# Autodesk Inventor assembly: GFRP_T2_09
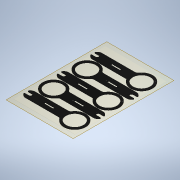
[picture p0: Inventor's stored thumbnail of the model, 180x180]
Saved by Autodesk Inventor 2020 (Build 240168000, 168)
## iProperties
Created: 2021-08-27
Part Number: GFRP_T2_09
Document SubType Name: Assembly
Designer: Masato
Author: Masato
## Documents named in this file (3)
- C:\Users\naoki\Documents\Inventor\CitBrains\git_clone\SUSTAINA_ver1_0\A_T2_175\SUSTAINA-OP\Cam\GFRP_T2_09.iam
- C:\Users\naoki\Documents\Inventor\CitBrains\git_clone\SUSTAINA_ver1_0\A_T2_175\SUSTAINA-OP\Cam\DisposableBoard.ipt
- C:\Users\naoki\Documents\Inventor\CitBrains\git_clone\SUSTAINA_ver1_0\A_T2_175\SUSTAINA-OP\UpperBody\Arm\ForeArm_outside_frame.ipt
## Components (6 placed, 2 different names)
1. DisposableBoard:1 — メイト:2, メイト:1, フラッシュ:1, フラッシュ:2, メイト:4, メイト:5, 角度:1, 正接:1, 正接:2, 正接:3, メイト:6, 正接:6
2. ForeArm_outside_frame:5 — メイト:6, 正接:5, 正接:6, 角度:3
3. ForeArm_outside_frame:1 — メイト:4, 角度:1, 角度:2, 正接:1, 正接:2, 正接:4
4. ForeArm_outside_frame:2 — メイト:5, 角度:2, 正接:3, 正接:4
5. ForeArm_outside_frame:3
6. ForeArm_outside_frame:4 — 正接:5, 角度:3
## Component patterns: (2 elements, first: ForeArm_outside_frame:1 + ForeArm_outside_frame:2)
## Relationships (16: Tangent 6, Mate 5, Angle 3, Flush 2)
- メイト:2 [Mate]: DisposableBoard:1
- メイト:1 [Mate]: DisposableBoard:1
- フラッシュ:1 [Flush]: DisposableBoard:1
- フラッシュ:2 [Flush]: DisposableBoard:1
- メイト:4 [Mate]: DisposableBoard:1 ↔ ForeArm_outside_frame:1
- メイト:5 [Mate]: DisposableBoard:1 ↔ ForeArm_outside_frame:2
- 角度:1 [Angle] (0 deg): DisposableBoard:1 ↔ ForeArm_outside_frame:1
- 角度:2 [Angle] (0 deg): ForeArm_outside_frame:1 ↔ ForeArm_outside_frame:2
- 正接:1 [Tangent] (2 mm): DisposableBoard:1 ↔ ForeArm_outside_frame:1
- 正接:2 [Tangent] (2 mm): DisposableBoard:1 ↔ ForeArm_outside_frame:1
- 正接:3 [Tangent] (2 mm): DisposableBoard:1 ↔ ForeArm_outside_frame:2
- 正接:4 [Tangent] (2.5 mm): ForeArm_outside_frame:1 ↔ ForeArm_outside_frame:2
- メイト:6 [Mate]: DisposableBoard:1 ↔ ForeArm_outside_frame:5
- 正接:5 [Tangent] (2.5 mm): ForeArm_outside_frame:5 ↔ ForeArm_outside_frame:4
- 正接:6 [Tangent] (2 mm): DisposableBoard:1 ↔ ForeArm_outside_frame:5
- 角度:3 [Angle] (0 deg): ForeArm_outside_frame:5 ↔ ForeArm_outside_frame:4
